# Autodesk Inventor assembly: LCD
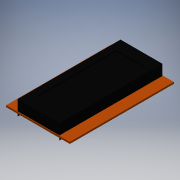
[picture p0: Inventor's stored thumbnail of the model, 180x180]
Saved by Autodesk Inventor 2016 (Build 200138000, 138)
## iProperties
Created: 2016-04-06
Part Number: LCD
Document SubType Name: Assembly
Designer: agmle
Author: agmle
## Documents named in this file (3)
- C:\Users\agmle\BitTorrent Sync\private\projects\Creekfleet_Timer\hardware\CAD\Main\LCD.iam
- C:\Users\agmle\BitTorrent Sync\private\projects\Creekfleet_Timer\hardware\CAD\Main\LCD_PCB.ipt
- C:\Users\agmle\BitTorrent Sync\private\projects\Creekfleet_Timer\hardware\CAD\Main\LCD_Screen.ipt
## Components (2 placed, 2 different names)
1. LCD_PCB:1 — Mate:1, Mate:2, Mate:3
2. LCD_Screen:1 — Mate:1, Mate:2, Mate:3
## Relationships (3: Mate 3)
- Mate:1: LCD_PCB:1 ↔ LCD_Screen:1
- Mate:2: LCD_PCB:1 ↔ LCD_Screen:1
- Mate:3: LCD_PCB:1 ↔ LCD_Screen:1
